# Autodesk Inventor assembly: B_beam
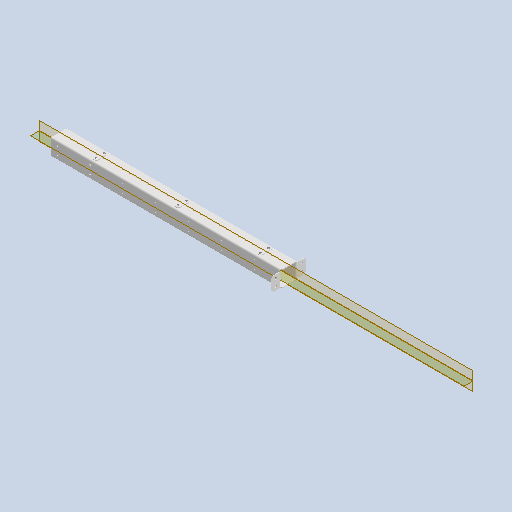
[picture p0: Inventor's stored thumbnail of the model, 512x512]
Saved by Autodesk Inventor 2025.2 (Build 292293000, 293)
## iProperties
Created: 2025-04-08
Part Number: B_beam
Document SubType Name: Assembly
Designer: Caspe
Author: Caspe
## Documents named in this file (5)
- C:\Users\Caspe\Documents\Semester 8\Project\Anomaly_Detection\Mechanical_Project\Inventor_project\B_beam.iam
- C:\Users\Caspe\Documents\Semester 8\Project\Anomaly_Detection\Mechanical_Project\Inventor_project\B_Beam.ipt
- C:\Users\Caspe\Documents\Semester 8\Project\Anomaly_Detection\Mechanical_Project\Inventor_project\A1_joiners.ipt
- C:\Users\Caspe\Documents\Inventor\Content Center Files\R2025\en-US\Blind Rivet GB_T 12615.1-2004\Blind Rivet GB_T 12615.1-2004 3.2 X 12.ipt
- C:\Users\Caspe\Documents\Semester 8\Project\Anomaly_Detection\Mechanical_Project\Inventor_project\Leg_press_parameters.xlsx
## Components (20 placed, 3 different names)
1. B_Beam:1 — Mate:1, Mate:2, Insert:2, Flush:1, Flush:2
2. B_Beam:2 — Mate:1, Mate:2, Insert:1
3. Blind Rivet GB/T 12615.1-2004 3.2 X 12:1 — Insert:3
4. Blind Rivet GB/T 12615.1-2004 3.2 X 12:2 — Insert:4
5. A1_joiners:1 — Insert:1, Insert:2, Insert:3, Insert:4
6. Blind Rivet GB/T 12615.1-2004 3.2 X 12:3
7. Blind Rivet GB/T 12615.1-2004 3.2 X 12:4
8. A1_joiners:2
9. Blind Rivet GB/T 12615.1-2004 3.2 X 12:11
10. Blind Rivet GB/T 12615.1-2004 3.2 X 12:12
11. A1_joiners:6
12. Blind Rivet GB/T 12615.1-2004 3.2 X 12:7
13. Blind Rivet GB/T 12615.1-2004 3.2 X 12:8
14. A1_joiners:4
15. Blind Rivet GB/T 12615.1-2004 3.2 X 12:9
16. Blind Rivet GB/T 12615.1-2004 3.2 X 12:10
17. A1_joiners:5
18. Blind Rivet GB/T 12615.1-2004 3.2 X 12:13
19. Blind Rivet GB/T 12615.1-2004 3.2 X 12:14
20. A1_joiners:7
## Component patterns: (2 elements), (3 elements, first: Blind Rivet GB/T 12615.1-2004 3.2 X 12:1 + Blind Rivet GB/T 12615.1-2004 3.2 X 12:2 + A1_joiners:1), Component Pattern 3:2 (3 elements)
## Relationships (10: Mate 4, Insert 4, Flush 2)
- Mate:1: B_Beam:1 ↔ B_Beam:2
- Mate:2: B_Beam:1 ↔ B_Beam:2
- Insert:1: B_Beam:2 ↔ A1_joiners:1
- Insert:2: B_Beam:1 ↔ A1_joiners:1
- Insert:3: Blind Rivet GB/T 12615.1-2004 3.2 X 12:1 ↔ A1_joiners:1
- Insert:4: Blind Rivet GB/T 12615.1-2004 3.2 X 12:2 ↔ A1_joiners:1
- Flush:1 (-25 mm): B_Beam:1
- Flush:2 (-25 mm): B_Beam:1
- Mate:3
- Mate:4
## Named parameters: A_length = 1000 mm, A_width = 50 mm, A_bend = 20 mm, A_connection_width = 40 mm, A_displacement = 500 mm, A_hole_height = 10 mm, A_hole_length = 40 mm, A_joint_diameter = 10 mm, A_height = 50 mm, A_joint_tolerance = 3 mm, l___________ = 0 mm, B_length = 700 mm, B_height = 50 mm, B_width = 50 mm, B_bend = 20 mm, B_connection_width = 40 mm, B_hole_height = 10 mm, B_hole_length = 40 mm, l__________ = 0 mm, C_length = 400 mm, C_width = 20 mm, C_height = 330 mm, l_________ = 0 mm, rivet_diameter = 4 mm, rivet_displacement = 250 mm, plate_thickness = 2 mm, l________ = 0 mm, B_hinge_holes_spacing = 50 mm, A_B_spacing = 2 mm, L_Piston_Bottom = 21 mm, L_Piston_Top = 25 mm
